# Autodesk Inventor assembly: Foam_wing
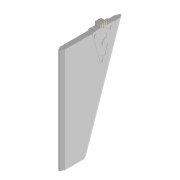
[picture p0: Inventor's stored thumbnail of the model, 180x180]
Saved by Autodesk Inventor 2022 (Build 260153000, 153)
## iProperties
Created: 2022-06-29
Part Number: Foam_wing
Document SubType Name: Assembly
Designer: dell
Author: dell
## Documents named in this file (6)
- D:\xxxx\Uni\Part IV\MECHENG_700\Part_IV_project_CAD\Bird_skeleton_prototypes\Wing_drone_V1\Foam_wing\Foam_wing.iam
- D:\xxxx\Uni\Part IV\MECHENG_700\Part_IV_project_CAD\Bird_skeleton_prototypes\Wing_drone_V1\Foam_wing\Foam_wing_mount.ipt
- D:\xxxx\Uni\Part IV\MECHENG_700\Part_IV_project_CAD\Bird_skeleton_prototypes\Wing_drone_V1\Foam_wing\Foam_wing_mount_clamp.ipt
- D:\xxxx\Uni\Part IV\MECHENG_700\Part_IV_project_CAD\Bird_skeleton_prototypes\Wing_drone_V1\Foam_wing\Foam_wing_mount_bolt.ipt
- D:\xxxx\Uni\Part IV\MECHENG_700\Part_IV_project_CAD\Bird_skeleton_prototypes\Wing_drone_V1\Foam_wing\Foam_wing_mount_washer.ipt
- D:\xxxx\Uni\Part IV\MECHENG_700\Part_IV_project_CAD\Bird_skeleton_prototypes\Wing_drone_V1\Foam_wing\Foam_wing_V2.ipt
## Components (12 placed, 5 different names)
1. Foam_wing_mount:1 — Mate:2, Mate:3, Mate:4, Mate:5, Mate:6, Mate:7, Mate:26, Mate:28
2. Foam_wing_mount_clamp:1 — Mate:2, Mate:3, Mate:4, Mate:16, Mate:20, Mate:24, Mate:27
3. Foam_wing_mount_clamp:2 — Mate:5, Mate:6, Mate:7, Mate:12, Mate:15, Mate:19, Mate:23
4. Foam_wing_mount_bolt:1 — Mate:9, Mate:12, Mate:13
5. Foam_wing_mount_bolt:2 — Mate:15, Mate:17
6. Foam_wing_mount_bolt:3 — Mate:23, Mate:25
7. Foam_wing_mount_bolt:4 — Mate:19, Mate:21
8. Foam_wing_mount_washer:2 — Mate:9, Mate:13
9. Foam_wing_mount_washer:3 — Mate:20, Mate:21
10. Foam_wing_mount_washer:4 — Mate:24, Mate:25
11. Foam_wing_mount_washer:5 — Mate:16, Mate:17
12. Foam_wing_V2:3 — Mate:26, Mate:27, Mate:28
## Relationships (21: Mate 21)
- Mate:2: Foam_wing_mount:1 ↔ Foam_wing_mount_clamp:1
- Mate:3: Foam_wing_mount:1 ↔ Foam_wing_mount_clamp:1
- Mate:4: Foam_wing_mount:1 ↔ Foam_wing_mount_clamp:1
- Mate:5: Foam_wing_mount:1 ↔ Foam_wing_mount_clamp:2
- Mate:6: Foam_wing_mount:1 ↔ Foam_wing_mount_clamp:2
- Mate:7: Foam_wing_mount:1 ↔ Foam_wing_mount_clamp:2
- Mate:9: Foam_wing_mount_bolt:1 ↔ Foam_wing_mount_washer:2
- Mate:12: Foam_wing_mount_clamp:2 ↔ Foam_wing_mount_bolt:1
- Mate:13: Foam_wing_mount_bolt:1 ↔ Foam_wing_mount_washer:2
- Mate:15: Foam_wing_mount_clamp:2 ↔ Foam_wing_mount_bolt:2
- Mate:16: Foam_wing_mount_clamp:1 ↔ Foam_wing_mount_washer:5
- Mate:17: Foam_wing_mount_bolt:2 ↔ Foam_wing_mount_washer:5
- Mate:19: Foam_wing_mount_clamp:2 ↔ Foam_wing_mount_bolt:4
- Mate:20: Foam_wing_mount_clamp:1 ↔ Foam_wing_mount_washer:3
- Mate:21: Foam_wing_mount_bolt:4 ↔ Foam_wing_mount_washer:3
- Mate:23: Foam_wing_mount_clamp:2 ↔ Foam_wing_mount_bolt:3
- Mate:24: Foam_wing_mount_clamp:1 ↔ Foam_wing_mount_washer:4
- Mate:25: Foam_wing_mount_bolt:3 ↔ Foam_wing_mount_washer:4
- Mate:26: Foam_wing_mount:1 ↔ Foam_wing_V2:3
- Mate:27: Foam_wing_mount_clamp:1 ↔ Foam_wing_V2:3
- Mate:28 (-240 mm): Foam_wing_mount:1 ↔ Foam_wing_V2:3
